# Autodesk Inventor assembly: 2016-01-27-RhinoRobotBasicFrame
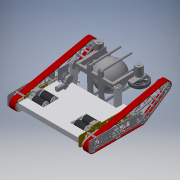
[picture p0: Inventor's stored thumbnail of the model, 180x180]
Saved by Autodesk Inventor 2016 SP1 (Build 200210100, 210)
## iProperties
Created: 2016-01-27
Part Number: 2016-01-27-RhinoRobotBasicFrame
Document SubType Name: Assembly
Designer: bbier
Sending System: Autodesk Inventor 2016
Preprocessor: ST-DEVELOPER v16.1
Title: C:\snobotics\CAD-Development\robSteele\SnoBotics2016\2016-01-27-RhinoRobot\2016-01-27-RhinoRobotBasicFrame.stp
Author: steele
## Documents named in this file (7)
- C:\snobotics\CAD-Development\robSteele\SnoBotics2016\Brian Bierman\2015-02-05\2016-01-27-RhinoRobotBasicFrame.iam
- C:\snobotics\CAD-Development\robSteele\SnoBotics2016\Brian Bierman\2015-02-05\x\am-3322+RhinoTrackDriveModule.iam
- C:\snobotics\CAD-Development\robSteele\SnoBotics2016\Brian Bierman\2015-02-05\x\am-3322+RhinoTrackDriveModule_MIR7.iam
- C:\snobotics\CAD-Development\robSteele\SnoBotics2016\Brian Bierman\2015-02-05\x\snoInsidePlate.ipt
- C:\snobotics\CAD-Development\robSteele\SnoBotics2016\Brian Bierman\2015-02-05\x\Assembly1.iam
- C:\snobotics\CAD-Development\robSteele\SnoBotics2016\Brian Bierman\2015-02-05\x\RhinoBottomFloorPlate03.ipt
- C:\snobotics\CAD-Development\robSteele\SnoBotics2016\Brian Bierman\2015-02-05\x\AM-2235.iam
## Components (6 placed, 6 different names)
1. am-3322+RhinoTrackDriveModule:1 [sub-assembly] — Flush:1, Flush:2, Mate:1
2. am-3322+RhinoTrackDriveModule_MIR7:1 [sub-assembly] — Flush:3, Flush:4, Mate:2
3. snoInsidePlate:1 — Flush:1, Flush:2, Mate:1, Flush:3, Flush:4, Mate:2, Mate:3, Mate:4, Mate:5, Mate:6, Flush:5, Mate:7
4. Assembly1:1 [sub-assembly] — Mate:3, Mate:4, Mate:5, Flush:6
5. RhinoBottomFloorPlate03:1 — Mate:6, Flush:5, Mate:7
6. AM-2235:1 [sub-assembly] — Flush:6
## Relationships (13: Mate 7, Flush 6)
- Flush:1: am-3322+RhinoTrackDriveModule:1 ↔ snoInsidePlate:1
- Flush:2: am-3322+RhinoTrackDriveModule:1 ↔ snoInsidePlate:1
- Mate:1: am-3322+RhinoTrackDriveModule:1 ↔ snoInsidePlate:1
- Flush:3: am-3322+RhinoTrackDriveModule_MIR7:1 ↔ snoInsidePlate:1
- Flush:4: am-3322+RhinoTrackDriveModule_MIR7:1 ↔ snoInsidePlate:1
- Mate:2: am-3322+RhinoTrackDriveModule_MIR7:1 ↔ snoInsidePlate:1
- Mate:3 (15.875 mm): snoInsidePlate:1 ↔ Assembly1:1
- Mate:4: snoInsidePlate:1 ↔ Assembly1:1
- Mate:5: snoInsidePlate:1 ↔ Assembly1:1
- Mate:6: snoInsidePlate:1 ↔ RhinoBottomFloorPlate03:1
- Flush:5: snoInsidePlate:1 ↔ RhinoBottomFloorPlate03:1
- Mate:7: snoInsidePlate:1 ↔ RhinoBottomFloorPlate03:1
- Flush:6: Assembly1:1 ↔ AM-2235:1
